# Autodesk Inventor assembly: Assemblyint
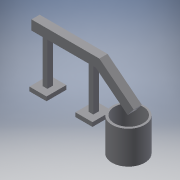
[picture p0: Inventor's stored thumbnail of the model, 180x180]
Saved by Autodesk Inventor 2019 (Build 230136000, 136)
## iProperties
Created: 2020-04-19
Part Number: Assemblyint
Document SubType Name: Assembly
Designer: dvg
Author: dvg
## Documents named in this file (3)
- C:\Users\dvg\Documents\Assemblyint.iam
- C:\Users\dvg\Documents\int.ipt
- C:\Users\dvg\Documents\int 3.ipt
## Components (3 placed, 2 different names)
1. int:1 — Mate:1, Mate:2
2. int 3:1 — Mate:1
3. int 3:2 — Mate:2
## Relationships (2: Mate 2)
- Mate:1: int:1 ↔ int 3:1
- Mate:2: int:1 ↔ int 3:2
